# Autodesk Inventor assembly: base_roulante_pmi
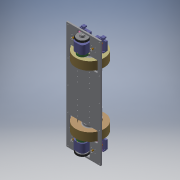
[picture p0: Inventor's stored thumbnail of the model, 180x180]
Saved by Autodesk Inventor 2019 (Build 230136000, 136)
## iProperties
Created: 2020-02-16
Part Number: base_roulante_pmi
Document SubType Name: Assembly
Designer: franc
Author: franc
## Documents named in this file (10)
- C:\Users\franc\Desktop\EsialRobotik\Mecanique\base_roulante\base_roulante_pmi.iam
- C:\Users\franc\Desktop\EsialRobotik\Mecanique\base_roulante\bloc_moteur.iam
- C:\Users\franc\Desktop\EsialRobotik\Mecanique\base_roulante\composants\capuchon_roulement.ipt
- C:\Users\franc\Desktop\EsialRobotik\Mecanique\base_roulante\composants\LM4UU.ipt
- C:\Users\franc\Desktop\EsialRobotik\Mecanique\base_roulante\axe_codeur.iam
- C:\Users\franc\Desktop\EsialRobotik\Mecanique\base_roulante\composants\support_codeur S65J.ipt
- C:\Users\franc\Desktop\EsialRobotik\Mecanique\base_roulante\socle_ammovible_pmi.ipt
- C:\Users\franc\Desktop\EsialRobotik\Mecanique\base_roulante\composants\Joint_torique_100mm.ipt
- C:\Users\franc\Desktop\EsialRobotik\Mecanique\base_roulante\composants\Roue_codeuse_100mm.ipt
- C:\Users\franc\Desktop\EsialRobotik\Mecanique\base_roulante\composants\Codeur_S25-J_Hengxiang.ipt
## Components (23 placed, 9 different names)
1. bloc_moteur:1 [sub-assembly] — Placage:45, Placage:46, Placage:47
2. bloc_moteur:2 [sub-assembly] — Placage:48, Placage:49, Placage:50
3. capuchon_roulement:1 — Placage:36, Placage:51, Placage:52, Placage:53
4. capuchon_roulement:2 — Placage:54, Placage:55, Placage:56
5. LM4UU:1 — Placage:60, Affleurement:2
6. LM4UU:2 — Placage:61, Affleurement:3
7. LM4UU:3 — Placage:25, Placage:58, Placage:59
8. LM4UU:4 — Placage:26, Placage:57, Affleurement:1
9. axe_codeur:1 [sub-assembly] — Placage:25, Placage:32, Placage:34
10. axe_codeur:2 [sub-assembly] — Placage:26, Placage:33, Placage:35
11. support_codeur S65J:1 — Placage:32, Placage:33, Placage:34, Placage:35, Placage:36, Placage:83, Placage:84, Placage:85
12. socle_ammovible_pmi:1 — Placage:45, Placage:46, Placage:47, Placage:48, Placage:49, Placage:50, Placage:51, Placage:52, Placage:53, Placage:54, Placage:55, Placage:56, Placage:57, Affleurement:1, Placage:58, Placage:59, Placage:60, Affleurement:2, Placage:61, Affleurement:3, Placage:62, Placage:63, Placage:64, Placage:65, Placage:66, Placage:67
13. axe_codeur:3 [sub-assembly] — Placage:71, Placage:73, Placage:75
14. axe_codeur:4 [sub-assembly] — Placage:72, Placage:74, Placage:76
15. capuchon_roulement:3 — Placage:65, Placage:66, Placage:67, Placage:71, Placage:77
16. capuchon_roulement:4 — Placage:62, Placage:63, Placage:64, Placage:72
17. support_codeur S65J:2 — Placage:73, Placage:74, Placage:75, Placage:76, Placage:77, Placage:80, Placage:81, Placage:82
18. Joint_torique_100mm:1 — Placage:78, Tangente:1
19. Joint_torique_100mm:2 — Placage:79, Tangente:2
20. Roue_codeuse_100mm:1 — Placage:78, Tangente:1, Placage:87, Affleurement:4
21. Roue_codeuse_100mm:2 — Placage:79, Tangente:2, Affleurement:5, Placage:88
22. Codeur_S25-J_Hengxiang:1 — Placage:80, Placage:81, Placage:82, Placage:87, Affleurement:4
23. Codeur_S25-J_Hengxiang:2 — Placage:83, Placage:84, Placage:85, Affleurement:5, Placage:88
## Relationships (54: Mate 47, Flush 5, Tangent 2)
- Placage:25 [Mate]: LM4UU:3 ↔ axe_codeur:1
- Placage:26 [Mate]: LM4UU:4 ↔ axe_codeur:2
- Placage:32 [Mate]: axe_codeur:1 ↔ support_codeur S65J:1
- Placage:33 [Mate]: axe_codeur:2 ↔ support_codeur S65J:1
- Placage:34 [Mate]: axe_codeur:1 ↔ support_codeur S65J:1
- Placage:35 [Mate]: axe_codeur:2 ↔ support_codeur S65J:1
- Placage:36 [Mate] (8 mm): capuchon_roulement:1 ↔ support_codeur S65J:1
- Placage:45 [Mate]: bloc_moteur:1 ↔ socle_ammovible_pmi:1
- Placage:46 [Mate]: bloc_moteur:1 ↔ socle_ammovible_pmi:1
- Placage:47 [Mate]: bloc_moteur:1 ↔ socle_ammovible_pmi:1
- Placage:48 [Mate]: bloc_moteur:2 ↔ socle_ammovible_pmi:1
- Placage:49 [Mate]: bloc_moteur:2 ↔ socle_ammovible_pmi:1
- Placage:50 [Mate]: bloc_moteur:2 ↔ socle_ammovible_pmi:1
- Placage:51 [Mate]: capuchon_roulement:1 ↔ socle_ammovible_pmi:1
- Placage:52 [Mate]: capuchon_roulement:1 ↔ socle_ammovible_pmi:1
- Placage:53 [Mate]: capuchon_roulement:1 ↔ socle_ammovible_pmi:1
- Placage:54 [Mate]: capuchon_roulement:2 ↔ socle_ammovible_pmi:1
- Placage:55 [Mate]: capuchon_roulement:2 ↔ socle_ammovible_pmi:1
- Placage:56 [Mate]: capuchon_roulement:2 ↔ socle_ammovible_pmi:1
- Placage:57 [Mate]: LM4UU:4 ↔ socle_ammovible_pmi:1
- Affleurement:1 [Flush]: LM4UU:4 ↔ socle_ammovible_pmi:1
- Placage:58 [Mate]: LM4UU:3 ↔ socle_ammovible_pmi:1
- Placage:59 [Mate]: LM4UU:3 ↔ socle_ammovible_pmi:1
- Placage:60 [Mate]: LM4UU:1 ↔ socle_ammovible_pmi:1
- Affleurement:2 [Flush]: LM4UU:1 ↔ socle_ammovible_pmi:1
- Placage:61 [Mate]: LM4UU:2 ↔ socle_ammovible_pmi:1
- Affleurement:3 [Flush]: LM4UU:2 ↔ socle_ammovible_pmi:1
- Placage:62 [Mate]: socle_ammovible_pmi:1 ↔ capuchon_roulement:4
- Placage:63 [Mate]: socle_ammovible_pmi:1 ↔ capuchon_roulement:4
- Placage:64 [Mate]: socle_ammovible_pmi:1 ↔ capuchon_roulement:4
- Placage:65 [Mate]: socle_ammovible_pmi:1 ↔ capuchon_roulement:3
- Placage:66 [Mate]: socle_ammovible_pmi:1 ↔ capuchon_roulement:3
- Placage:67 [Mate]: socle_ammovible_pmi:1 ↔ capuchon_roulement:3
- Placage:71 [Mate]: axe_codeur:3 ↔ capuchon_roulement:3
- Placage:72 [Mate]: axe_codeur:4 ↔ capuchon_roulement:4
- Placage:73 [Mate]: axe_codeur:3 ↔ support_codeur S65J:2
- Placage:74 [Mate]: axe_codeur:4 ↔ support_codeur S65J:2
- Placage:75 [Mate]: axe_codeur:3 ↔ support_codeur S65J:2
- Placage:76 [Mate]: axe_codeur:4 ↔ support_codeur S65J:2
- Placage:77 [Mate] (8 mm): capuchon_roulement:3 ↔ support_codeur S65J:2
- Placage:78 [Mate]: Joint_torique_100mm:1 ↔ Roue_codeuse_100mm:1
- Tangente:1: Joint_torique_100mm:1 ↔ Roue_codeuse_100mm:1
- Placage:79 [Mate]: Joint_torique_100mm:2 ↔ Roue_codeuse_100mm:2
- Tangente:2: Joint_torique_100mm:2 ↔ Roue_codeuse_100mm:2
- Placage:80 [Mate]: support_codeur S65J:2 ↔ Codeur_S25-J_Hengxiang:1
- Placage:81 [Mate]: support_codeur S65J:2 ↔ Codeur_S25-J_Hengxiang:1
- Placage:82 [Mate]: support_codeur S65J:2 ↔ Codeur_S25-J_Hengxiang:1
- Placage:83 [Mate]: support_codeur S65J:1 ↔ Codeur_S25-J_Hengxiang:2
- Placage:84 [Mate]: support_codeur S65J:1 ↔ Codeur_S25-J_Hengxiang:2
- Placage:85 [Mate]: support_codeur S65J:1 ↔ Codeur_S25-J_Hengxiang:2
- Placage:87 [Mate]: Roue_codeuse_100mm:1 ↔ Codeur_S25-J_Hengxiang:1
- Affleurement:4 [Flush]: Roue_codeuse_100mm:1 ↔ Codeur_S25-J_Hengxiang:1
- Affleurement:5 [Flush]: Roue_codeuse_100mm:2 ↔ Codeur_S25-J_Hengxiang:2
- Placage:88 [Mate]: Roue_codeuse_100mm:2 ↔ Codeur_S25-J_Hengxiang:2
